# Autodesk Inventor assembly: A2017_T4_03
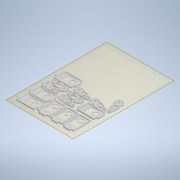
[picture p0: Inventor's stored thumbnail of the model, 180x180]
Saved by Autodesk Inventor 2020 (Build 240168000, 168)
## iProperties
Created: 2021-08-27
Part Number: A2017_T4_03
Document SubType Name: Assembly
Designer: Masato
Author: Masato
## Documents named in this file (4)
- C:\Inventor\SUSTAINA-OP\Cam\A2017_T4_03.iam
- C:\Inventor\SUSTAINA-OP\Cam\DisposableBoard.ipt
- C:\Inventor\SUSTAINA-OP\UpperBody\Trunk\Trunk_servo_bottom_frame.ipt
- C:\Inventor\SUSTAINA-OP\LowerBody\Ankle\Ankle_side_pitch_frame.ipt
## Components (15 placed, 3 different names)
1. DisposableBoard:1 — メイト:2, メイト:1, フラッシュ:1, フラッシュ:2, メイト:4, メイト:5, メイト:6, メイト:7, メイト:9, フラッシュ:3, フラッシュ:4, メイト:16, フラッシュ:11, フラッシュ:12, メイト:17, メイト:18, メイト:19, メイト:20, 正接:1, メイト:27, メイト:28, メイト:29, メイト:31, フラッシュ:13
2. Trunk_servo_bottom_frame:1 — メイト:4, メイト:11, フラッシュ:6, メイト:21, 正接:2
3. Trunk_servo_bottom_frame:2 — メイト:6, フラッシュ:8, フラッシュ:9, メイト:12, メイト:13
4. Trunk_servo_bottom_frame:3 — メイト:7, フラッシュ:3, フラッシュ:4, メイト:11, フラッシュ:6, フラッシュ:7, メイト:14
5. Trunk_servo_bottom_frame:4 — メイト:5, フラッシュ:7, フラッシュ:8, メイト:13, メイト:14, メイト:24
6. Trunk_servo_bottom_frame:6 — メイト:9, フラッシュ:9, メイト:12, メイト:26
7. Trunk_servo_bottom_frame:7 — メイト:16, フラッシュ:11, フラッシュ:12, メイト:23, 正接:5
8. Ankle_side_pitch_frame:1 — メイト:17, メイト:22, メイト:23, 正接:3
9. Ankle_side_pitch_frame:2 — メイト:18, メイト:21, 正接:1, メイト:22
10. Ankle_side_pitch_frame:3 — メイト:20, メイト:24, 正接:2, メイト:25
11. Ankle_side_pitch_frame:4 — メイト:19, メイト:25, 正接:3, 正接:4, メイト:30
12. Trunk_servo_bottom_frame:8 — メイト:26, メイト:27, 正接:4, メイト:32, 正接:7
13. Ankle_side_pitch_frame:5 — メイト:28, メイト:30, 正接:5, 正接:6
14. Ankle_side_pitch_frame:6 — メイト:29, 正接:6, メイト:32
15. Ankle_side_pitch_frame:7 — メイト:31, フラッシュ:13, 正接:7
## Relationships (46: Mate 28, Flush 11, Tangent 7)
- メイト:2 [Mate]: DisposableBoard:1
- メイト:1 [Mate]: DisposableBoard:1
- フラッシュ:1 [Flush]: DisposableBoard:1
- フラッシュ:2 [Flush]: DisposableBoard:1
- メイト:4 [Mate]: DisposableBoard:1 ↔ Trunk_servo_bottom_frame:1
- メイト:5 [Mate]: DisposableBoard:1 ↔ Trunk_servo_bottom_frame:4
- メイト:6 [Mate]: DisposableBoard:1 ↔ Trunk_servo_bottom_frame:2
- メイト:7 [Mate]: DisposableBoard:1 ↔ Trunk_servo_bottom_frame:3
- メイト:9 [Mate]: DisposableBoard:1 ↔ Trunk_servo_bottom_frame:6
- フラッシュ:3 [Flush] (1.5 mm): DisposableBoard:1 ↔ Trunk_servo_bottom_frame:3
- フラッシュ:4 [Flush] (1.5 mm): DisposableBoard:1 ↔ Trunk_servo_bottom_frame:3
- メイト:11 [Mate] (2.5 mm): Trunk_servo_bottom_frame:1 ↔ Trunk_servo_bottom_frame:3
- フラッシュ:6 [Flush]: Trunk_servo_bottom_frame:1 ↔ Trunk_servo_bottom_frame:3
- フラッシュ:7 [Flush]: Trunk_servo_bottom_frame:3 ↔ Trunk_servo_bottom_frame:4
- フラッシュ:8 [Flush]: Trunk_servo_bottom_frame:2 ↔ Trunk_servo_bottom_frame:4
- フラッシュ:9 [Flush]: Trunk_servo_bottom_frame:2 ↔ Trunk_servo_bottom_frame:6
- メイト:12 [Mate] (2.5 mm): Trunk_servo_bottom_frame:2 ↔ Trunk_servo_bottom_frame:6
- メイト:13 [Mate] (2.5 mm): Trunk_servo_bottom_frame:2 ↔ Trunk_servo_bottom_frame:4
- メイト:14 [Mate] (2.5 mm): Trunk_servo_bottom_frame:3 ↔ Trunk_servo_bottom_frame:4
- メイト:16 [Mate]: DisposableBoard:1 ↔ Trunk_servo_bottom_frame:7
- フラッシュ:11 [Flush] (125 mm): DisposableBoard:1 ↔ Trunk_servo_bottom_frame:7
- フラッシュ:12 [Flush] (1.5 mm): DisposableBoard:1 ↔ Trunk_servo_bottom_frame:7
- メイト:17 [Mate]: DisposableBoard:1 ↔ Ankle_side_pitch_frame:1
- メイト:18 [Mate]: DisposableBoard:1 ↔ Ankle_side_pitch_frame:2
- メイト:19 [Mate]: DisposableBoard:1 ↔ Ankle_side_pitch_frame:4
- メイト:20 [Mate]: DisposableBoard:1 ↔ Ankle_side_pitch_frame:3
- メイト:21 [Mate] (2.5 mm): Trunk_servo_bottom_frame:1 ↔ Ankle_side_pitch_frame:2
- 正接:1 [Tangent] (1.5 mm): DisposableBoard:1 ↔ Ankle_side_pitch_frame:2
- メイト:22 [Mate] (2.5 mm): Ankle_side_pitch_frame:1 ↔ Ankle_side_pitch_frame:2
- メイト:23 [Mate] (2.5 mm): Trunk_servo_bottom_frame:7 ↔ Ankle_side_pitch_frame:1
- メイト:24 [Mate] (2.5 mm): Trunk_servo_bottom_frame:4 ↔ Ankle_side_pitch_frame:3
- 正接:2 [Tangent] (2.5 mm): Trunk_servo_bottom_frame:1 ↔ Ankle_side_pitch_frame:3
- メイト:25 [Mate] (2.5 mm): Ankle_side_pitch_frame:3 ↔ Ankle_side_pitch_frame:4
- 正接:3 [Tangent] (2.5 mm): Ankle_side_pitch_frame:1 ↔ Ankle_side_pitch_frame:4
- メイト:26 [Mate] (3.5 mm): Trunk_servo_bottom_frame:6 ↔ Trunk_servo_bottom_frame:8
- メイト:27 [Mate]: DisposableBoard:1 ↔ Trunk_servo_bottom_frame:8
- 正接:4 [Tangent] (4.5 mm): Ankle_side_pitch_frame:4 ↔ Trunk_servo_bottom_frame:8
- メイト:28 [Mate]: DisposableBoard:1 ↔ Ankle_side_pitch_frame:5
- メイト:29 [Mate]: DisposableBoard:1 ↔ Ankle_side_pitch_frame:6
- メイト:30 [Mate] (2.5 mm): Ankle_side_pitch_frame:4 ↔ Ankle_side_pitch_frame:5
- 正接:5 [Tangent] (2.5 mm): Trunk_servo_bottom_frame:7 ↔ Ankle_side_pitch_frame:5
- 正接:6 [Tangent] (2.5 mm): Ankle_side_pitch_frame:5 ↔ Ankle_side_pitch_frame:6
- メイト:31 [Mate]: DisposableBoard:1 ↔ Ankle_side_pitch_frame:7
- メイト:32 [Mate] (0.5 mm): Trunk_servo_bottom_frame:8 ↔ Ankle_side_pitch_frame:6
- フラッシュ:13 [Flush] (1.5 mm): DisposableBoard:1 ↔ Ankle_side_pitch_frame:7
- 正接:7 [Tangent] (5 mm): Trunk_servo_bottom_frame:8 ↔ Ankle_side_pitch_frame:7
